# Autodesk Inventor assembly: Hand Kwik-Mount
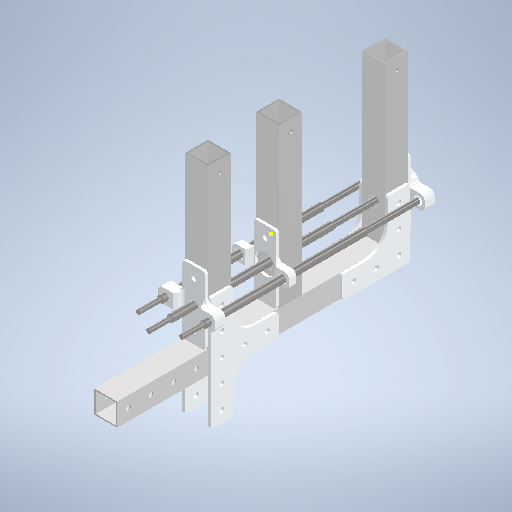
[picture p0: Inventor's stored thumbnail of the model, 512x512]
Saved by Autodesk Inventor 2025.1 (Build 291241020, 241B)
## iProperties
Created: 2024-01-20
Part Number: Hand Kwik-Mount
Document SubType Name: Assembly
Designer: aidan
Author: aidan
## Documents named in this file (9)
- C:\Users\aidan\Documents\BehrendURCMechanical\CAD\Chassis V3\Robotic Claw\CH - Hand W Standard Gussets.iam
- C:\Users\aidan\OneDrive\Documents\Inventor\Content Center Files\am-4158 1IN Tee Gusset.ipt
- C:\Users\aidan\OneDrive\Documents\Inventor\Content Center Files\am-3860 90 Gusset REV2.ipt
- C:\Users\aidan\Documents\BehrendURCMechanical\CAD\Chassis V3\Robotic Claw\Tube Finger.ipt
- C:\Users\aidan\Documents\BehrendURCMechanical\CAD\Chassis V3\Robotic Claw\Lead Nut Holder Mk2.ipt
- C:\Users\aidan\Documents\BehrendURCMechanical\CAD\Chassis V3\Robotic Claw\Guide Rod Holder.ipt
- C:\Users\aidan\Documents\BehrendURCMechanical\CAD\Chassis V3\Robotic Claw\Finger Base.ipt
- C:\Users\aidan\Documents\BehrendURCMechanical\CAD\Chassis V3\Robotic Claw\Lead_Shaft.ipt
- C:\Users\aidan\Documents\BehrendURCMechanical\CAD\Chassis V3\Robotic Claw\Bearing Holder.ipt
## Components (14 placed, 8 different names)
1. am-3860 90 Gusset REV2:1
2. am-3860 90 Gusset REV2:2
3. Tube Finger:1
4. Tube Finger:2 — Mate:1, Mate:2, Mate:3
5. Lead Nut Holder Mk2:1 — Mate:3
6. Tube Finger:3
7. Finger Base:1 — Mate:1, Mate:2
8. am-4158 1IN Tee Gusset:1
9. am-4158 1IN Tee Gusset:2
10. Guide Rod Holder:2
11. Lead_Shaft:1
12. Lead_Shaft:2
13. Lead_Shaft:3
14. Bearing Holder:1
## Relationships (3: Mate 3)
- Mate:1: Tube Finger:2 ↔ Finger Base:1
- Mate:2: Tube Finger:2 ↔ Finger Base:1
- Mate:3: Tube Finger:2 ↔ Lead Nut Holder Mk2:1
